# Autodesk Inventor assembly: romi-chassis-kit
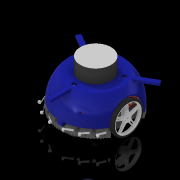
[picture p0: Inventor's stored thumbnail of the model, 180x180]
Saved by Autodesk Inventor 2020.3 (Build 243373000, 373)
## iProperties
Created: 2017-06-08
Part Number: romi-chassis-kit
Description: STEP AP214
Document SubType Name: Assembly
Designer: Britt
Sending System: SolidWorks 2016
Preprocessor: SwSTEP 2.0
Title: romi-chassis-kit.step
Revision Number: ANY
## Documents named in this file (10)
- C:\Users\david\Desktop\BrittVentorLISAT\romi-chassis-kit.iam
- C:\Users\david\Desktop\BrittVentorLISAT\chassis.ipt
- C:\Users\david\Desktop\BrittVentorLISAT\battery-cover.ipt
- C:\Users\david\Desktop\BrittVentorLISAT\wheel.ipt
- C:\Users\david\Desktop\BrittVentorLISAT\front-caster.ipt
- C:\Users\david\Desktop\BrittVentorLISAT\RobotHoedje.ipt
- C:\Users\david\Desktop\BrittVentorLISAT\Speakertje.ipt
- C:\Users\david\Desktop\BrittVentorLISAT\romi-ti-rslk-max-bumper-switch-assembly.ipt
- C:\Users\david\Desktop\BrittVentorLISAT\ti-rslk-max-chassis-board-v1.0.ipt
- C:\Users\david\Desktop\BrittVentorLISAT\Blokje.ipt
## Components (11 placed, 10 different names)
1. chassis_1 — Mate:1, Mate:4, Mate:5, Mate:6, Mate:7, Mate:8, Mate:10, Mate:11
2. battery-cover_2
3. wheel_3
4. wheel_4
5. front-caster_5
6. RobotHoedje:1 — Mate:1, Mate:2, Mate:3, Mate:10, Mate:11
7. Speakertje:1 — Mate:2, Mate:3
8. romi-ti-rslk-max-bumper-switch-assembly:1 — Mate:4
9. romi-ti-rslk-max-bumper-switch-assembly:2 — Mate:5
10. ti-rslk-max-chassis-board-v1.0:1 — Mate:6, Mate:7, Mate:8, Mate:9, Flush:1
11. Blokje:1 — Mate:9, Flush:1
## Relationships (12: Mate 11, Flush 1)
- Mate:1: chassis_1 ↔ RobotHoedje:1
- Mate:2: RobotHoedje:1 ↔ Speakertje:1
- Mate:3: RobotHoedje:1 ↔ Speakertje:1
- Mate:4: chassis_1 ↔ romi-ti-rslk-max-bumper-switch-assembly:1
- Mate:5: chassis_1 ↔ romi-ti-rslk-max-bumper-switch-assembly:2
- Mate:6: chassis_1 ↔ ti-rslk-max-chassis-board-v1.0:1
- Mate:7: chassis_1 ↔ ti-rslk-max-chassis-board-v1.0:1
- Mate:8: chassis_1 ↔ ti-rslk-max-chassis-board-v1.0:1
- Mate:9: ti-rslk-max-chassis-board-v1.0:1 ↔ Blokje:1
- Flush:1: ti-rslk-max-chassis-board-v1.0:1 ↔ Blokje:1
- Mate:10: chassis_1 ↔ RobotHoedje:1
- Mate:11: chassis_1 ↔ RobotHoedje:1
